# Autodesk Inventor assembly: Goldberg Assembly
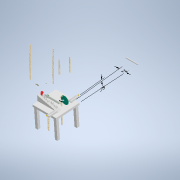
[picture p0: Inventor's stored thumbnail of the model, 180x180]
Saved by Autodesk Inventor 2021 (Build 250183000, 183)
## iProperties
Created: 2021-02-17
Part Number: Goldberg Assembly
Document SubType Name: Assembly
Designer: david
Author: david
## Documents named in this file (17)
- C:\Users\david\OneDrive\Documents\Inventor\Goldberg Assembly.iam
- C:\Users\david\OneDrive\Documents\Inventor\Tabl 12x12.ipt
- C:\Users\david\OneDrive\Documents\Inventor\Ball Ramp - Goldberg.ipt
- C:\Users\david\OneDrive\Documents\Inventor\Ball sphere - goldberg.ipt
- C:\Users\david\OneDrive\Documents\Inventor\Domino ramp.ipt
- C:\Users\david\OneDrive\Documents\Inventor\Domino.ipt
- C:\Users\david\OneDrive\Documents\Inventor\Cup- red.ipt
- C:\Users\david\OneDrive\Documents\Inventor\Inventor_2013_VEX_KOP_-_Imperial\Imperial\Motion\36 Tooth Gear.ipt
- C:\Users\david\OneDrive\Documents\Inventor\Inventor_2013_VEX_KOP_-_Imperial\Imperial\Motion\Shaft 2 inch.ipt
- C:\Users\david\OneDrive\Documents\Inventor\Inventor_2013_VEX_KOP_-_Imperial\Imperial\Motion\High Strength 6 Tooth Sprocket.ipt
- C:\Users\david\OneDrive\Documents\Inventor\Inventor_2013_VEX_KOP_-_Imperial\Imperial\Motion\High Strength 30 Tooth Sprocket.ipt
- C:\Users\david\OneDrive\Documents\Inventor\Inventor_2013_VEX_KOP_-_Imperial\Imperial\Motion\Chain Link.ipt
- C:\Users\david\OneDrive\Documents\Inventor\Inventor_2013_VEX_KOP_-_Imperial\Imperial\Motion\High Strength Chain Link.ipt
- C:\Users\david\OneDrive\Documents\Inventor\Inventor_2013_VEX_KOP_-_Imperial\Imperial\Motion\Tank Tread Traction Link.ipt
- C:\Users\david\OneDrive\Documents\Inventor\Inventor_2013_VEX_KOP_-_Imperial\Imperial\Structure\Chassis Bumper 15 Hole.ipt
- C:\Users\david\OneDrive\Documents\Inventor\Inventor_2013_VEX_KOP_-_Imperial\Imperial\Motion\Bearing Flat.ipt
- C:\Users\david\OneDrive\Documents\stick.ipt
## Components (228 placed, 16 different names)
1. Tabl 12x12:1 — Mate:1, Flush:1, Mate:2, Mate:3, Flush:2, Flush:3, Mate:22, Flush:4
2. Ball Ramp - Goldberg:1 — Mate:3, Mate:4, Flush:2, Tangent:1
3. Ball Ramp - Goldberg:2 — Mate:2, Tangent:2
4. Ball sphere - goldberg:1 — Tangent:1
5. Ball sphere - goldberg:2 — Tangent:2
6. Domino ramp:1 — Mate:1, Flush:1, Mate:4, Flush:3, Mate:5, Mate:6, Mate:7, Mate:8, Mate:9, Mate:10, Mate:11, Mate:12, Mate:13, Mate:14, Mate:15, Mate:16, Mate:17, Mate:18, Mate:20, Mate:21
7. Domino:1 — Mate:5
8. Domino:2 — Mate:7
9. Domino:3 — Mate:8
10. Domino:4 — Mate:6
11. Domino:5 — Mate:9
12. Domino:6 — Mate:10
13. Domino:7 — Mate:12
14. Domino:8 — Mate:15
15. Domino:9 — Mate:14
16. Domino:10 — Mate:11
17. Domino:11 — Mate:13
18. Cup- red:1 — Mate:16
19. Domino:12 — Mate:17
20. Domino:13 — Mate:18
21. 36 Tooth Gear:1 — Insert:81
22. Shaft 2 inch:1 — Mate:20, Insert:81, Insert:82
23. High Strength 6 Tooth Sprocket:1 — Mate:19, Insert:2, Insert:82
24. High Strength 30 Tooth Sprocket:1 — Mate:25, Mate:26, Mate:27, Mate:28, Mate:29
25. Chain Link:1
26. High Strength Chain Link:1 — Insert:1, Insert:2, Insert:276
27. High Strength Chain Link:3 — Insert:1, Mate:19
28. Tank Tread Traction Link:1
29. High Strength Chain Link:4 — Insert:9, Insert:10
30. High Strength Chain Link:10 — Insert:6, Insert:7, Insert:8, Insert:18
31. High Strength Chain Link:15 — Insert:11
32. High Strength Chain Link:21 — Insert:6, Insert:7, Insert:8, Insert:9
33. High Strength Chain Link:28 — Insert:10, Insert:11
34. High Strength Chain Link:31
35. High Strength Chain Link:32 — Insert:32
36. High Strength Chain Link:33 — Insert:18
37. High Strength Chain Link:34
38. High Strength Chain Link:35
39. High Strength Chain Link:36
40. High Strength Chain Link:37
41. High Strength Chain Link:38 — Insert:32
42. High Strength Chain Link:39
43. High Strength Chain Link:40
44. High Strength Chain Link:41
45. High Strength Chain Link:42 — Insert:110
46. High Strength Chain Link:43
47. High Strength Chain Link:44
48. High Strength Chain Link:45
49. High Strength Chain Link:46
50. High Strength Chain Link:47
51. High Strength Chain Link:48
52. High Strength Chain Link:49
53. High Strength Chain Link:50
54. High Strength Chain Link:51
55. High Strength Chain Link:52
56. High Strength Chain Link:53
57. High Strength Chain Link:54
58. High Strength Chain Link:55
59. High Strength Chain Link:56
60. High Strength Chain Link:57
61. High Strength Chain Link:58
62. High Strength Chain Link:59
63. High Strength Chain Link:60
64. High Strength Chain Link:61
65. High Strength Chain Link:62
66. High Strength Chain Link:63
67. High Strength Chain Link:64
68. High Strength Chain Link:65
69. High Strength Chain Link:66
70. High Strength Chain Link:67
71. High Strength Chain Link:68
72. High Strength Chain Link:69
73. High Strength Chain Link:70
74. High Strength Chain Link:71
75. High Strength Chain Link:72
76. High Strength Chain Link:73
77. High Strength Chain Link:74
78. High Strength Chain Link:75
79. High Strength Chain Link:76
80. High Strength Chain Link:77
81. High Strength Chain Link:78
82. High Strength Chain Link:79
83. High Strength Chain Link:80
84. High Strength Chain Link:81
85. High Strength Chain Link:82 — Insert:110
86. High Strength Chain Link:83
87. High Strength Chain Link:84
88. High Strength Chain Link:85
89. High Strength Chain Link:86
90. High Strength Chain Link:87
91. High Strength Chain Link:88
92. High Strength Chain Link:89
93. High Strength Chain Link:90
94. High Strength Chain Link:91
95. High Strength Chain Link:92
96. High Strength Chain Link:93
97. High Strength Chain Link:94
98. High Strength Chain Link:95
99. High Strength Chain Link:96
100. High Strength Chain Link:97
101. High Strength Chain Link:98
102. High Strength Chain Link:99
103. High Strength Chain Link:100
104. High Strength Chain Link:101
105. High Strength Chain Link:102
106. High Strength Chain Link:103
107. High Strength Chain Link:104
108. High Strength Chain Link:105
109. High Strength Chain Link:106
110. High Strength Chain Link:107
111. High Strength Chain Link:108
112. High Strength Chain Link:109
113. High Strength Chain Link:110
114. High Strength Chain Link:111
115. High Strength Chain Link:112
116. High Strength Chain Link:113
117. High Strength Chain Link:114
118. High Strength Chain Link:115
119. High Strength Chain Link:116
120. High Strength Chain Link:117
121. High Strength Chain Link:118
122. High Strength Chain Link:119
123. High Strength Chain Link:120
124. High Strength Chain Link:121
125. High Strength Chain Link:122
126. High Strength Chain Link:123
127. High Strength Chain Link:124
128. High Strength Chain Link:125
129. High Strength Chain Link:126
130. High Strength Chain Link:127
131. High Strength Chain Link:128
132. High Strength Chain Link:129
133. High Strength Chain Link:130
134. High Strength Chain Link:131
135. High Strength Chain Link:132
136. High Strength Chain Link:133
137. High Strength Chain Link:134
138. High Strength Chain Link:135
139. High Strength Chain Link:136 — Insert:276
140. High Strength Chain Link:137
141. High Strength Chain Link:138
142. High Strength Chain Link:139
143. High Strength Chain Link:140
144. High Strength Chain Link:141
145. High Strength Chain Link:142
146. High Strength Chain Link:143
147. High Strength Chain Link:144
148. High Strength Chain Link:145
149. High Strength Chain Link:146
150. High Strength Chain Link:147
151. High Strength Chain Link:148
152. High Strength Chain Link:149
153. High Strength Chain Link:150
154. High Strength Chain Link:151
155. High Strength Chain Link:152
156. High Strength Chain Link:153
157. High Strength Chain Link:154
158. High Strength Chain Link:155
159. High Strength Chain Link:156
160. High Strength Chain Link:157
161. High Strength Chain Link:158
162. High Strength Chain Link:159
163. High Strength Chain Link:160
164. High Strength Chain Link:161
165. High Strength Chain Link:162
166. High Strength Chain Link:163
167. High Strength Chain Link:164
168. High Strength Chain Link:165
169. High Strength Chain Link:166
170. High Strength Chain Link:167
171. High Strength Chain Link:168
172. High Strength Chain Link:169
173. High Strength Chain Link:170
174. High Strength Chain Link:171
175. High Strength Chain Link:172
176. High Strength Chain Link:173
177. High Strength Chain Link:174
178. High Strength Chain Link:175
179. High Strength Chain Link:176
180. High Strength Chain Link:177
181. High Strength Chain Link:178
182. High Strength Chain Link:179
183. High Strength Chain Link:180
184. High Strength Chain Link:181
185. High Strength Chain Link:182
186. High Strength Chain Link:183
187. High Strength Chain Link:184
188. High Strength Chain Link:185
189. High Strength Chain Link:186
190. High Strength Chain Link:187
191. High Strength Chain Link:188
192. High Strength Chain Link:189
193. High Strength Chain Link:190
194. High Strength Chain Link:191
195. High Strength Chain Link:192
196. High Strength Chain Link:193
197. High Strength Chain Link:194
198. High Strength Chain Link:195
199. High Strength Chain Link:196
200. High Strength Chain Link:197
201. High Strength Chain Link:198
202. High Strength Chain Link:199
203. High Strength Chain Link:200
204. High Strength Chain Link:201
205. High Strength Chain Link:202
206. High Strength Chain Link:203
207. High Strength Chain Link:204
208. High Strength Chain Link:205
209. High Strength Chain Link:206
210. High Strength Chain Link:207
211. High Strength Chain Link:208
212. High Strength Chain Link:209
213. High Strength Chain Link:210
214. High Strength Chain Link:211 — Mate:28
215. High Strength Chain Link:212
216. High Strength Chain Link:213 — Mate:29, Mate:30
217. High Strength Chain Link:214
218. High Strength Chain Link:215 — Mate:27
219. High Strength Chain Link:216
220. High Strength Chain Link:217 — Mate:30
221. High Strength Chain Link:218
222. High Strength Chain Link:219 — Mate:26
223. Chassis Bumper 15 Hole:1 — Mate:21, Mate:22, Flush:4, Mate:23, Mate:24, Flush:5
224. Shaft 2 inch:2 — Mate:23, Mate:24, Flush:5, Insert:277
225. Bearing Flat:1 — Insert:277, Mate:25
226. stick:1
227. stick:2
228. stick:3
## Relationships (311: Insert 274, Mate 30, Flush 5, Tangent 2)
- Mate:1: Tabl 12x12:1 ↔ Domino ramp:1
- Flush:1 (203.2 mm): Tabl 12x12:1 ↔ Domino ramp:1
- Mate:2: Tabl 12x12:1 ↔ Ball Ramp - Goldberg:2
- Mate:3: Tabl 12x12:1 ↔ Ball Ramp - Goldberg:1
- Mate:4: Ball Ramp - Goldberg:1 ↔ Domino ramp:1
- Flush:2 (50.8 mm): Tabl 12x12:1 ↔ Ball Ramp - Goldberg:1
- Flush:3: Tabl 12x12:1 ↔ Domino ramp:1
- Mate:5: Domino ramp:1 ↔ Domino:1
- Mate:6: Domino ramp:1 ↔ Domino:4
- Mate:7: Domino ramp:1 ↔ Domino:2
- Mate:8: Domino ramp:1 ↔ Domino:3
- Mate:9: Domino ramp:1 ↔ Domino:5
- Mate:10: Domino ramp:1 ↔ Domino:6
- Mate:11: Domino ramp:1 ↔ Domino:10
- Mate:12: Domino ramp:1 ↔ Domino:7
- Mate:13: Domino ramp:1 ↔ Domino:11
- Mate:14: Domino ramp:1 ↔ Domino:9
- Mate:15: Domino ramp:1 ↔ Domino:8
- Mate:16: Domino ramp:1 ↔ Cup- red:1
- Mate:17: Domino ramp:1 ↔ Domino:12
- Mate:18: Domino ramp:1 ↔ Domino:13
- Tangent:1: Ball Ramp - Goldberg:1 ↔ Ball sphere - goldberg:1
- Tangent:2: Ball Ramp - Goldberg:2 ↔ Ball sphere - goldberg:2
- Insert:1: High Strength Chain Link:1 ↔ High Strength Chain Link:3
- Mate:19: High Strength 6 Tooth Sprocket:1 ↔ High Strength Chain Link:3
- Insert:2: High Strength 6 Tooth Sprocket:1 ↔ High Strength Chain Link:1
- Insert:6: High Strength Chain Link:10 ↔ High Strength Chain Link:21
- Insert:7: High Strength Chain Link:10 ↔ High Strength Chain Link:21
- Insert:8: High Strength Chain Link:10 ↔ High Strength Chain Link:21
- Insert:9: High Strength Chain Link:4 ↔ High Strength Chain Link:21
- Insert:10: High Strength Chain Link:4 ↔ High Strength Chain Link:28
- Insert:11: High Strength Chain Link:15 ↔ High Strength Chain Link:28
- [Insert]: High Strength Chain Link:32 ↔ High Strength Chain Link:34
- [Insert]: High Strength Chain Link:32 ↔ High Strength Chain Link:34
- [Insert]: High Strength Chain Link:32 ↔ High Strength Chain Link:34
- [Insert]: High Strength Chain Link:31 ↔ High Strength Chain Link:34
- [Insert]: High Strength Chain Link:31 ↔ High Strength Chain Link:35
- [Insert]: High Strength Chain Link:33 ↔ High Strength Chain Link:35
- Insert:18: High Strength Chain Link:10 ↔ High Strength Chain Link:33
- [Insert]: High Strength Chain Link:37 ↔ High Strength Chain Link:39
- [Insert]: High Strength Chain Link:37 ↔ High Strength Chain Link:39
- [Insert]: High Strength Chain Link:37 ↔ High Strength Chain Link:39
- [Insert]: High Strength Chain Link:36 ↔ High Strength Chain Link:39
- [Insert]: High Strength Chain Link:36 ↔ High Strength Chain Link:40
- [Insert]: High Strength Chain Link:38 ↔ High Strength Chain Link:40
- [Insert]: High Strength Chain Link:42 ↔ High Strength Chain Link:44
- [Insert]: High Strength Chain Link:42 ↔ High Strength Chain Link:44
- [Insert]: High Strength Chain Link:42 ↔ High Strength Chain Link:44
- [Insert]: High Strength Chain Link:41 ↔ High Strength Chain Link:44
- [Insert]: High Strength Chain Link:41 ↔ High Strength Chain Link:45
- [Insert]: High Strength Chain Link:43 ↔ High Strength Chain Link:45
- [Insert]: High Strength Chain Link:37 ↔ High Strength Chain Link:43
- Insert:32: High Strength Chain Link:32 ↔ High Strength Chain Link:38
- [Insert]: High Strength Chain Link:46 ↔ High Strength Chain Link:47
- [Insert]: High Strength Chain Link:46 ↔ High Strength Chain Link:47
- [Insert]: High Strength Chain Link:46 ↔ High Strength Chain Link:47
- [Insert]: High Strength Chain Link:49 ↔ High Strength Chain Link:51
- [Insert]: High Strength Chain Link:49 ↔ High Strength Chain Link:51
- [Insert]: High Strength Chain Link:49 ↔ High Strength Chain Link:51
- [Insert]: High Strength Chain Link:48 ↔ High Strength Chain Link:51
- [Insert]: High Strength Chain Link:48 ↔ High Strength Chain Link:52
- [Insert]: High Strength Chain Link:50 ↔ High Strength Chain Link:52
- [Insert]: High Strength Chain Link:46 ↔ High Strength Chain Link:50
- [Insert]: High Strength Chain Link:54 ↔ High Strength Chain Link:56
- [Insert]: High Strength Chain Link:54 ↔ High Strength Chain Link:56
- [Insert]: High Strength Chain Link:54 ↔ High Strength Chain Link:56
- [Insert]: High Strength Chain Link:53 ↔ High Strength Chain Link:56
- [Insert]: High Strength Chain Link:53 ↔ High Strength Chain Link:57
- [Insert]: High Strength Chain Link:55 ↔ High Strength Chain Link:57
- [Insert]: High Strength Chain Link:59 ↔ High Strength Chain Link:61
- [Insert]: High Strength Chain Link:59 ↔ High Strength Chain Link:61
- [Insert]: High Strength Chain Link:59 ↔ High Strength Chain Link:61
- [Insert]: High Strength Chain Link:58 ↔ High Strength Chain Link:61
- [Insert]: High Strength Chain Link:58 ↔ High Strength Chain Link:62
- [Insert]: High Strength Chain Link:60 ↔ High Strength Chain Link:62
- [Insert]: High Strength Chain Link:54 ↔ High Strength Chain Link:60
- [Insert]: High Strength Chain Link:49 ↔ High Strength Chain Link:55
- [Insert]: High Strength Chain Link:63 ↔ High Strength Chain Link:64
- [Insert]: High Strength Chain Link:63 ↔ High Strength Chain Link:64
- [Insert]: High Strength Chain Link:63 ↔ High Strength Chain Link:64
- [Insert]: High Strength Chain Link:66 ↔ High Strength Chain Link:68
- [Insert]: High Strength Chain Link:66 ↔ High Strength Chain Link:68
- [Insert]: High Strength Chain Link:66 ↔ High Strength Chain Link:68
- [Insert]: High Strength Chain Link:65 ↔ High Strength Chain Link:68
- [Insert]: High Strength Chain Link:65 ↔ High Strength Chain Link:69
- [Insert]: High Strength Chain Link:67 ↔ High Strength Chain Link:69
- [Insert]: High Strength Chain Link:63 ↔ High Strength Chain Link:67
- [Insert]: High Strength Chain Link:71 ↔ High Strength Chain Link:73
- [Insert]: High Strength Chain Link:71 ↔ High Strength Chain Link:73
- [Insert]: High Strength Chain Link:71 ↔ High Strength Chain Link:73
- [Insert]: High Strength Chain Link:70 ↔ High Strength Chain Link:73
- [Insert]: High Strength Chain Link:70 ↔ High Strength Chain Link:74
- [Insert]: High Strength Chain Link:72 ↔ High Strength Chain Link:74
- [Insert]: High Strength Chain Link:76 ↔ High Strength Chain Link:78
- [Insert]: High Strength Chain Link:76 ↔ High Strength Chain Link:78
- [Insert]: High Strength Chain Link:76 ↔ High Strength Chain Link:78
- [Insert]: High Strength Chain Link:75 ↔ High Strength Chain Link:78
- [Insert]: High Strength Chain Link:75 ↔ High Strength Chain Link:79
- [Insert]: High Strength Chain Link:77 ↔ High Strength Chain Link:79
- [Insert]: High Strength Chain Link:71 ↔ High Strength Chain Link:77
- [Insert]: High Strength Chain Link:66 ↔ High Strength Chain Link:72
- Mate:20: Domino ramp:1 ↔ Shaft 2 inch:1
- Insert:81 (-31.75 mm): 36 Tooth Gear:1 ↔ Shaft 2 inch:1
- Insert:82 (-6.35 mm): Shaft 2 inch:1 ↔ High Strength 6 Tooth Sprocket:1
- [Insert]: High Strength Chain Link:81 ↔ High Strength Chain Link:83
- [Insert]: High Strength Chain Link:81 ↔ High Strength Chain Link:83
- [Insert]: High Strength Chain Link:81 ↔ High Strength Chain Link:83
- [Insert]: High Strength Chain Link:80 ↔ High Strength Chain Link:83
- [Insert]: High Strength Chain Link:80 ↔ High Strength Chain Link:84
- [Insert]: High Strength Chain Link:82 ↔ High Strength Chain Link:84
- [Insert]: High Strength Chain Link:86 ↔ High Strength Chain Link:88
- [Insert]: High Strength Chain Link:86 ↔ High Strength Chain Link:88
- [Insert]: High Strength Chain Link:86 ↔ High Strength Chain Link:88
- [Insert]: High Strength Chain Link:85 ↔ High Strength Chain Link:88
- [Insert]: High Strength Chain Link:85 ↔ High Strength Chain Link:89
- [Insert]: High Strength Chain Link:87 ↔ High Strength Chain Link:89
- [Insert]: High Strength Chain Link:81 ↔ High Strength Chain Link:87
- [Insert]: High Strength Chain Link:91 ↔ High Strength Chain Link:93
- [Insert]: High Strength Chain Link:91 ↔ High Strength Chain Link:93
- [Insert]: High Strength Chain Link:91 ↔ High Strength Chain Link:93
- [Insert]: High Strength Chain Link:90 ↔ High Strength Chain Link:93
- [Insert]: High Strength Chain Link:90 ↔ High Strength Chain Link:94
- [Insert]: High Strength Chain Link:92 ↔ High Strength Chain Link:94
- [Insert]: High Strength Chain Link:96 ↔ High Strength Chain Link:98
- [Insert]: High Strength Chain Link:96 ↔ High Strength Chain Link:98
- [Insert]: High Strength Chain Link:96 ↔ High Strength Chain Link:98
- [Insert]: High Strength Chain Link:95 ↔ High Strength Chain Link:98
- [Insert]: High Strength Chain Link:95 ↔ High Strength Chain Link:99
- [Insert]: High Strength Chain Link:97 ↔ High Strength Chain Link:99
- [Insert]: High Strength Chain Link:91 ↔ High Strength Chain Link:97
- [Insert]: High Strength Chain Link:86 ↔ High Strength Chain Link:92
- Insert:110: High Strength Chain Link:42 ↔ High Strength Chain Link:82
- [Insert]: High Strength Chain Link:101 ↔ High Strength Chain Link:103
- [Insert]: High Strength Chain Link:101 ↔ High Strength Chain Link:103
- [Insert]: High Strength Chain Link:101 ↔ High Strength Chain Link:103
- [Insert]: High Strength Chain Link:100 ↔ High Strength Chain Link:103
- [Insert]: High Strength Chain Link:100 ↔ High Strength Chain Link:104
- [Insert]: High Strength Chain Link:102 ↔ High Strength Chain Link:104
- [Insert]: High Strength Chain Link:106 ↔ High Strength Chain Link:108
- [Insert]: High Strength Chain Link:106 ↔ High Strength Chain Link:108
- [Insert]: High Strength Chain Link:106 ↔ High Strength Chain Link:108
- [Insert]: High Strength Chain Link:105 ↔ High Strength Chain Link:108
- [Insert]: High Strength Chain Link:105 ↔ High Strength Chain Link:109
- [Insert]: High Strength Chain Link:107 ↔ High Strength Chain Link:109
- [Insert]: High Strength Chain Link:101 ↔ High Strength Chain Link:107
- [Insert]: High Strength Chain Link:111 ↔ High Strength Chain Link:113
- [Insert]: High Strength Chain Link:111 ↔ High Strength Chain Link:113
- [Insert]: High Strength Chain Link:111 ↔ High Strength Chain Link:113
- [Insert]: High Strength Chain Link:110 ↔ High Strength Chain Link:113
- [Insert]: High Strength Chain Link:110 ↔ High Strength Chain Link:114
- [Insert]: High Strength Chain Link:112 ↔ High Strength Chain Link:114
- [Insert]: High Strength Chain Link:116 ↔ High Strength Chain Link:118
- [Insert]: High Strength Chain Link:116 ↔ High Strength Chain Link:118
- [Insert]: High Strength Chain Link:116 ↔ High Strength Chain Link:118
- [Insert]: High Strength Chain Link:115 ↔ High Strength Chain Link:118
- [Insert]: High Strength Chain Link:115 ↔ High Strength Chain Link:119
- [Insert]: High Strength Chain Link:117 ↔ High Strength Chain Link:119
- [Insert]: High Strength Chain Link:111 ↔ High Strength Chain Link:117
- [Insert]: High Strength Chain Link:106 ↔ High Strength Chain Link:112
- [Insert]: High Strength Chain Link:121 ↔ High Strength Chain Link:123
- [Insert]: High Strength Chain Link:121 ↔ High Strength Chain Link:123
- [Insert]: High Strength Chain Link:121 ↔ High Strength Chain Link:123
- [Insert]: High Strength Chain Link:120 ↔ High Strength Chain Link:123
- [Insert]: High Strength Chain Link:120 ↔ High Strength Chain Link:124
- [Insert]: High Strength Chain Link:122 ↔ High Strength Chain Link:124
- [Insert]: High Strength Chain Link:126 ↔ High Strength Chain Link:128
- [Insert]: High Strength Chain Link:126 ↔ High Strength Chain Link:128
- [Insert]: High Strength Chain Link:126 ↔ High Strength Chain Link:128
- [Insert]: High Strength Chain Link:125 ↔ High Strength Chain Link:128
- [Insert]: High Strength Chain Link:125 ↔ High Strength Chain Link:129
- [Insert]: High Strength Chain Link:127 ↔ High Strength Chain Link:129
- [Insert]: High Strength Chain Link:121 ↔ High Strength Chain Link:127
- [Insert]: High Strength Chain Link:131 ↔ High Strength Chain Link:133
- [Insert]: High Strength Chain Link:131 ↔ High Strength Chain Link:133
- [Insert]: High Strength Chain Link:131 ↔ High Strength Chain Link:133
- [Insert]: High Strength Chain Link:130 ↔ High Strength Chain Link:133
- [Insert]: High Strength Chain Link:130 ↔ High Strength Chain Link:134
- [Insert]: High Strength Chain Link:132 ↔ High Strength Chain Link:134
- [Insert]: High Strength Chain Link:136 ↔ High Strength Chain Link:138
- [Insert]: High Strength Chain Link:136 ↔ High Strength Chain Link:138
- [Insert]: High Strength Chain Link:136 ↔ High Strength Chain Link:138
- [Insert]: High Strength Chain Link:135 ↔ High Strength Chain Link:138
- [Insert]: High Strength Chain Link:135 ↔ High Strength Chain Link:139
- [Insert]: High Strength Chain Link:137 ↔ High Strength Chain Link:139
- [Insert]: High Strength Chain Link:131 ↔ High Strength Chain Link:137
- [Insert]: High Strength Chain Link:126 ↔ High Strength Chain Link:132
- [Insert]: High Strength Chain Link:116 ↔ High Strength Chain Link:122
- [Insert]: High Strength Chain Link:141 ↔ High Strength Chain Link:143
- [Insert]: High Strength Chain Link:141 ↔ High Strength Chain Link:143
- [Insert]: High Strength Chain Link:141 ↔ High Strength Chain Link:143
- [Insert]: High Strength Chain Link:140 ↔ High Strength Chain Link:143
- [Insert]: High Strength Chain Link:140 ↔ High Strength Chain Link:144
- [Insert]: High Strength Chain Link:142 ↔ High Strength Chain Link:144
- [Insert]: High Strength Chain Link:146 ↔ High Strength Chain Link:148
- [Insert]: High Strength Chain Link:146 ↔ High Strength Chain Link:148
- [Insert]: High Strength Chain Link:146 ↔ High Strength Chain Link:148
- [Insert]: High Strength Chain Link:145 ↔ High Strength Chain Link:148
- [Insert]: High Strength Chain Link:145 ↔ High Strength Chain Link:149
- [Insert]: High Strength Chain Link:147 ↔ High Strength Chain Link:149
- [Insert]: High Strength Chain Link:141 ↔ High Strength Chain Link:147
- [Insert]: High Strength Chain Link:151 ↔ High Strength Chain Link:153
- [Insert]: High Strength Chain Link:151 ↔ High Strength Chain Link:153
- [Insert]: High Strength Chain Link:151 ↔ High Strength Chain Link:153
- [Insert]: High Strength Chain Link:150 ↔ High Strength Chain Link:153
- [Insert]: High Strength Chain Link:150 ↔ High Strength Chain Link:154
- [Insert]: High Strength Chain Link:152 ↔ High Strength Chain Link:154
- [Insert]: High Strength Chain Link:156 ↔ High Strength Chain Link:158
- [Insert]: High Strength Chain Link:156 ↔ High Strength Chain Link:158
- [Insert]: High Strength Chain Link:156 ↔ High Strength Chain Link:158
- [Insert]: High Strength Chain Link:155 ↔ High Strength Chain Link:158
- [Insert]: High Strength Chain Link:155 ↔ High Strength Chain Link:159
- [Insert]: High Strength Chain Link:157 ↔ High Strength Chain Link:159
- [Insert]: High Strength Chain Link:151 ↔ High Strength Chain Link:157
- [Insert]: High Strength Chain Link:146 ↔ High Strength Chain Link:152
- [Insert]: High Strength Chain Link:161 ↔ High Strength Chain Link:163
- [Insert]: High Strength Chain Link:161 ↔ High Strength Chain Link:163
- [Insert]: High Strength Chain Link:161 ↔ High Strength Chain Link:163
- [Insert]: High Strength Chain Link:160 ↔ High Strength Chain Link:163
- [Insert]: High Strength Chain Link:160 ↔ High Strength Chain Link:164
- [Insert]: High Strength Chain Link:162 ↔ High Strength Chain Link:164
- [Insert]: High Strength Chain Link:166 ↔ High Strength Chain Link:168
- [Insert]: High Strength Chain Link:166 ↔ High Strength Chain Link:168
- [Insert]: High Strength Chain Link:166 ↔ High Strength Chain Link:168
- [Insert]: High Strength Chain Link:165 ↔ High Strength Chain Link:168
- [Insert]: High Strength Chain Link:165 ↔ High Strength Chain Link:169
- [Insert]: High Strength Chain Link:167 ↔ High Strength Chain Link:169
- [Insert]: High Strength Chain Link:161 ↔ High Strength Chain Link:167
- [Insert]: High Strength Chain Link:171 ↔ High Strength Chain Link:173
- [Insert]: High Strength Chain Link:171 ↔ High Strength Chain Link:173
- [Insert]: High Strength Chain Link:171 ↔ High Strength Chain Link:173
- [Insert]: High Strength Chain Link:170 ↔ High Strength Chain Link:173
- [Insert]: High Strength Chain Link:170 ↔ High Strength Chain Link:174
- [Insert]: High Strength Chain Link:172 ↔ High Strength Chain Link:174
- [Insert]: High Strength Chain Link:176 ↔ High Strength Chain Link:178
- [Insert]: High Strength Chain Link:176 ↔ High Strength Chain Link:178
- [Insert]: High Strength Chain Link:176 ↔ High Strength Chain Link:178
- [Insert]: High Strength Chain Link:175 ↔ High Strength Chain Link:178
- [Insert]: High Strength Chain Link:175 ↔ High Strength Chain Link:179
- [Insert]: High Strength Chain Link:177 ↔ High Strength Chain Link:179
- [Insert]: High Strength Chain Link:171 ↔ High Strength Chain Link:177
- [Insert]: High Strength Chain Link:166 ↔ High Strength Chain Link:172
- [Insert]: High Strength Chain Link:156 ↔ High Strength Chain Link:162
- [Insert]: High Strength Chain Link:181 ↔ High Strength Chain Link:183
- [Insert]: High Strength Chain Link:181 ↔ High Strength Chain Link:183
- [Insert]: High Strength Chain Link:181 ↔ High Strength Chain Link:183
- [Insert]: High Strength Chain Link:180 ↔ High Strength Chain Link:183
- [Insert]: High Strength Chain Link:180 ↔ High Strength Chain Link:184
- [Insert]: High Strength Chain Link:182 ↔ High Strength Chain Link:184
- [Insert]: High Strength Chain Link:186 ↔ High Strength Chain Link:188
- [Insert]: High Strength Chain Link:186 ↔ High Strength Chain Link:188
- [Insert]: High Strength Chain Link:186 ↔ High Strength Chain Link:188
- [Insert]: High Strength Chain Link:185 ↔ High Strength Chain Link:188
- [Insert]: High Strength Chain Link:185 ↔ High Strength Chain Link:189
- [Insert]: High Strength Chain Link:187 ↔ High Strength Chain Link:189
- [Insert]: High Strength Chain Link:181 ↔ High Strength Chain Link:187
- [Insert]: High Strength Chain Link:191 ↔ High Strength Chain Link:193
- [Insert]: High Strength Chain Link:191 ↔ High Strength Chain Link:193
- [Insert]: High Strength Chain Link:191 ↔ High Strength Chain Link:193
- [Insert]: High Strength Chain Link:190 ↔ High Strength Chain Link:193
- [Insert]: High Strength Chain Link:190 ↔ High Strength Chain Link:194
- [Insert]: High Strength Chain Link:192 ↔ High Strength Chain Link:194
- [Insert]: High Strength Chain Link:196 ↔ High Strength Chain Link:198
- [Insert]: High Strength Chain Link:196 ↔ High Strength Chain Link:198
- [Insert]: High Strength Chain Link:196 ↔ High Strength Chain Link:198
- [Insert]: High Strength Chain Link:195 ↔ High Strength Chain Link:198
- [Insert]: High Strength Chain Link:195 ↔ High Strength Chain Link:199
- [Insert]: High Strength Chain Link:197 ↔ High Strength Chain Link:199
- [Insert]: High Strength Chain Link:191 ↔ High Strength Chain Link:197
- [Insert]: High Strength Chain Link:186 ↔ High Strength Chain Link:192
- [Insert]: High Strength Chain Link:201 ↔ High Strength Chain Link:203
- [Insert]: High Strength Chain Link:201 ↔ High Strength Chain Link:203
- [Insert]: High Strength Chain Link:201 ↔ High Strength Chain Link:203
- [Insert]: High Strength Chain Link:200 ↔ High Strength Chain Link:203
- [Insert]: High Strength Chain Link:200 ↔ High Strength Chain Link:204
- [Insert]: High Strength Chain Link:202 ↔ High Strength Chain Link:204
- [Insert]: High Strength Chain Link:206 ↔ High Strength Chain Link:208
- [Insert]: High Strength Chain Link:206 ↔ High Strength Chain Link:208
- [Insert]: High Strength Chain Link:206 ↔ High Strength Chain Link:208
- [Insert]: High Strength Chain Link:205 ↔ High Strength Chain Link:208
- [Insert]: High Strength Chain Link:205 ↔ High Strength Chain Link:209
- [Insert]: High Strength Chain Link:207 ↔ High Strength Chain Link:209
- [Insert]: High Strength Chain Link:201 ↔ High Strength Chain Link:207
- [Insert]: High Strength Chain Link:211 ↔ High Strength Chain Link:213
- [Insert]: High Strength Chain Link:211 ↔ High Strength Chain Link:213
- [Insert]: High Strength Chain Link:211 ↔ High Strength Chain Link:213
- [Insert]: High Strength Chain Link:210 ↔ High Strength Chain Link:213
- [Insert]: High Strength Chain Link:210 ↔ High Strength Chain Link:214
- [Insert]: High Strength Chain Link:212 ↔ High Strength Chain Link:214
- [Insert]: High Strength Chain Link:216 ↔ High Strength Chain Link:218
- [Insert]: High Strength Chain Link:216 ↔ High Strength Chain Link:218
- [Insert]: High Strength Chain Link:216 ↔ High Strength Chain Link:218
- [Insert]: High Strength Chain Link:215 ↔ High Strength Chain Link:218
- [Insert]: High Strength Chain Link:215 ↔ High Strength Chain Link:219
- [Insert]: High Strength Chain Link:217 ↔ High Strength Chain Link:219
- [Insert]: High Strength Chain Link:211 ↔ High Strength Chain Link:217
- [Insert]: High Strength Chain Link:206 ↔ High Strength Chain Link:212
- [Insert]: High Strength Chain Link:196 ↔ High Strength Chain Link:202
- Insert:276: High Strength Chain Link:1 ↔ High Strength Chain Link:136
- Mate:21: Domino ramp:1 ↔ Chassis Bumper 15 Hole:1
- Mate:22 (50.8 mm): Tabl 12x12:1 ↔ Chassis Bumper 15 Hole:1
- Flush:4 (76.2 mm): Tabl 12x12:1 ↔ Chassis Bumper 15 Hole:1
- Mate:23: Chassis Bumper 15 Hole:1 ↔ Shaft 2 inch:2
- Mate:24: Chassis Bumper 15 Hole:1 ↔ Shaft 2 inch:2
- Flush:5 (-12.7 mm): Chassis Bumper 15 Hole:1 ↔ Shaft 2 inch:2
- Insert:277 (-12.7 mm): Shaft 2 inch:2 ↔ Bearing Flat:1
- Mate:25: High Strength 30 Tooth Sprocket:1 ↔ Bearing Flat:1
- Mate:26: High Strength 30 Tooth Sprocket:1 ↔ High Strength Chain Link:219
- Mate:27: High Strength 30 Tooth Sprocket:1 ↔ High Strength Chain Link:215
- Mate:28: High Strength 30 Tooth Sprocket:1 ↔ High Strength Chain Link:211
- Mate:29: High Strength 30 Tooth Sprocket:1 ↔ High Strength Chain Link:213
- Mate:30: High Strength Chain Link:213 ↔ High Strength Chain Link:217
## Named parameters: d46_d44 = 0 mm, d47_d45 = 0 mm, d48_d40 = 0 mm, d49_d41 = 0 mm, d50_d42 = 0 mm, d51_d43 = 0 mm, d53_d44 = 0 mm, d54_d45 = 0 mm, d55_d46_d44 = 0 mm, d56_d47_d45 = 0 mm, d57_d48_d40 = 0 mm, d58_d49_d41 = 0 mm, d59_d50_d42 = 0 mm, d60_d51_d43 = 0 mm, d61_d52 = 0 mm, d62_d40 = 0 mm, d63_d41 = 0 mm, d64_d42 = 0 mm, d65_d43 = 0 mm, d67_d46_d44 = 0 mm, d68_d47_d45 = 0 mm, d69_d48_d40 = 0 mm, d70_d49_d41 = 0 mm, d71_d50_d42 = 0 mm, d72_d51_d43 = 0 mm, d73_d52 = 0 mm, d74_d53_d44 = 0 mm, d75_d54_d45 = 0 mm, d76_d55_d46_d44 = 0 mm, d77_d56_d47_d45 = 0 mm, d78_d57_d48_d40 = 0 mm, d79_d58_d49_d41 = 0 mm, d80_d59_d50_d42 = 0 mm, d81_d60_d51_d43 = 0 mm, d82_d61_d52 = 0 mm, d83_d62_d40 = 0 mm, d84_d63_d41 = 0 mm, d85_d64_d42 = 0 mm, d86_d65_d43 = 0 mm, d87_d40 = 0 mm, d88_d41 = 0 mm, d89_d42 = 0 mm, d90_d66 = 0 mm, d91_d67_d46_d44 = 0 mm, d92_d68_d47_d45 = 0 mm, d93_d69_d48_d40 = 0 mm, d94_d70_d49_d41 = 0 mm, d95_d71_d50_d42 = 0 mm, d96_d72_d51_d43 = 0 mm, d97_d73_d52 = 0 mm, d98_d74_d53_d44 = 0 mm, d99_d75_d54_d45 = 0 mm, d100_d76_d55_d46_d44 = 0 mm, d101_d77_d56_d47_d45 = 0 mm, d102_d78_d57_d48_d40 = 0 mm, d103_d79_d58_d49_d41 = 0 mm, d104_d80_d59_d50_d42 = 0 mm, d105_d81_d60_d51_d43 = 0 mm, d106_d82_d61_d52 = 0 mm, d107_d83_d62_d40 = 0 mm, d108_d84_d63_d41 = 0 mm, d109_d85_d64_d42 = 0 mm, d110_d86_d65_d43 = 0 mm, d111_d87_d40 = 0 mm, d112_d88_d41 = 0 mm, d113_d89_d42 = 0 mm, d114_d90_d66 = 0 mm, d118_d44 = 0 mm, d119_d45 = 0 mm, d120_d46_d44 = 0 mm, d121_d47_d45 = 0 mm, d122_d48_d40 = 0 mm, d123_d49_d41 = 0 mm, d124_d50_d42 = 0 mm, d125_d51_d43 = 0 mm, d126_d52 = 0 mm, d127_d53_d44 = 0 mm, d128_d54_d45 = 0 mm, d129_d55_d46_d44 = 0 mm, d130_d56_d47_d45 = 0 mm, d131_d57_d48_d40 = 0 mm, d132_d58_d49_d41 = 0 mm, d133_d59_d50_d42 = 0 mm, d134_d60_d51_d43 = 0 mm, d135_d61_d52 = 0 mm, d136_d62_d40 = 0 mm, d137_d63_d41 = 0 mm, d138_d64_d42 = 0 mm, d139_d65_d43 = 0 mm, d140_d40 = 0 mm, d141_d41 = 0 mm, d142_d42 = 0 mm, d143_d43 = 0 mm, d144_d66 = 0 mm, d146_d145 = 0 mm, d147_d44 = 0 mm, d148_d45 = 0 mm, d149_d46_d44 = 0 mm, d150_d47_d45 = 0 mm, d151_d48_d40 = 0 mm, d152_d49_d41 = 0 mm, d153_d50_d42 = 0 mm, d154_d51_d43 = 0 mm, d155_d52 = 0 mm, d156_d53_d44 = 0 mm, d157_d54_d45 = 0 mm, d158_d55_d46_d44 = 0 mm, d159_d56_d47_d45 = 0 mm, d160_d57_d48_d40 = 0 mm, d161_d58_d49_d41 = 0 mm, d162_d59_d50_d42 = 0 mm, d163_d60_d51_d43 = 0 mm, d164_d61_d52 = 0 mm, d165_d62_d40 = 0 mm, d166_d63_d41 = 0 mm, d167_d64_d42 = 0 mm, d168_d65_d43 = 0 mm, d169_d40 = 0 mm, d170_d41 = 0 mm, d171_d42 = 0 mm, d172_d43 = 0 mm, d173_d118_d44 = 0 mm, d174_d119_d45 = 0 mm, d175_d120_d46_d44 = 0 mm, d176_d121_d47_d45 = 0 mm, d177_d122_d48_d40 = 0 mm, d178_d123_d49_d41 = 0 mm, d179_d124_d50_d42 = 0 mm, d180_d125_d51_d43 = 0 mm, d181_d126_d52 = 0 mm, d182_d127_d53_d44 = 0 mm, d183_d128_d54_d45 = 0 mm, d184_d129_d55_d46_d44 = 0 mm, d185_d130_d56_d47_d45 = 0 mm, d186_d131_d57_d48_d40 = 0 mm, d187_d132_d58_d49_d41 = 0 mm, d188_d133_d59_d50_d42 = 0 mm, d189_d134_d60_d51_d43 = 0 mm, d190_d135_d61_d52 = 0 mm, d191_d136_d62_d40 = 0 mm, d192_d137_d63_d41 = 0 mm, d193_d138_d64_d42 = 0 mm, d194_d139_d65_d43 = 0 mm, d195_d140_d40 = 0 mm, d196_d141_d41 = 0 mm, d197_d142_d42 = 0 mm, d198_d143_d43 = 0 mm, d199_d144_d66 = 0 mm, d200_d66 = 0 mm, d201_d145 = 0 mm, d202_d44 = 0 mm, d203_d45 = 0 mm, d204_d46_d44 = 0 mm, d205_d47_d45 = 0 mm, d206_d48_d40 = 0 mm, d207_d49_d41 = 0 mm, d208_d50_d42 = 0 mm, d209_d51_d43 = 0 mm, d210_d52 = 0 mm, d211_d53_d44 = 0 mm, d212_d54_d45 = 0 mm, d213_d55_d46_d44 = 0 mm, d214_d56_d47_d45 = 0 mm, d215_d57_d48_d40 = 0 mm, d216_d58_d49_d41 = 0 mm, d217_d59_d50_d42 = 0 mm, d218_d60_d51_d43 = 0 mm, d219_d61_d52 = 0 mm, d220_d62_d40 = 0 mm, d221_d63_d41 = 0 mm, d222_d64_d42 = 0 mm, d223_d65_d43 = 0 mm, d224_d40 = 0 mm, d225_d41 = 0 mm, d226_d42 = 0 mm, d227_d43 = 0 mm, d228_d118_d44 = 0 mm, d229_d119_d45 = 0 mm, d230_d120_d46_d44 = 0 mm, d231_d121_d47_d45 = 0 mm, d232_d122_d48_d40 = 0 mm, d233_d123_d49_d41 = 0 mm, d234_d124_d50_d42 = 0 mm, d235_d125_d51_d43 = 0 mm, d236_d126_d52 = 0 mm, d237_d127_d53_d44 = 0 mm, d238_d128_d54_d45 = 0 mm, d239_d129_d55_d46_d44 = 0 mm, d240_d130_d56_d47_d45 = 0 mm, d241_d131_d57_d48_d40 = 0 mm, d242_d132_d58_d49_d41 = 0 mm, d243_d133_d59_d50_d42 = 0 mm, d244_d134_d60_d51_d43 = 0 mm, d245_d135_d61_d52 = 0 mm, d246_d136_d62_d40 = 0 mm, d247_d137_d63_d41 = 0 mm, d248_d138_d64_d42 = 0 mm, d249_d139_d65_d43 = 0 mm, d250_d140_d40 = 0 mm, d251_d141_d41 = 0 mm, d252_d142_d42 = 0 mm, d253_d143_d43 = 0 mm, d254_d144_d66 = 0 mm, d255_d66 = 0 mm, d256_d145 = 0 mm, d257_d44 = 0 mm, d258_d45 = 0 mm, d259_d46_d44 = 0 mm, d260_d47_d45 = 0 mm, d261_d48_d40 = 0 mm, d262_d49_d41 = 0 mm, d263_d50_d42 = 0 mm, d264_d51_d43 = 0 mm, d265_d52 = 0 mm, d266_d53_d44 = 0 mm, d267_d54_d45 = 0 mm, d268_d55_d46_d44 = 0 mm, d269_d56_d47_d45 = 0 mm, d270_d57_d48_d40 = 0 mm, d271_d58_d49_d41 = 0 mm, d272_d59_d50_d42 = 0 mm, d273_d60_d51_d43 = 0 mm, d274_d61_d52 = 0 mm, d275_d62_d40 = 0 mm, d276_d63_d41 = 0 mm, d277_d64_d42 = 0 mm, d278_d65_d43 = 0 mm, d279_d40 = 0 mm, d280_d41 = 0 mm, d281_d42 = 0 mm, d282_d43 = 0 mm, d283_d118_d44 = 0 mm, d284_d119_d45 = 0 mm, d285_d120_d46_d44 = 0 mm, d286_d121_d47_d45 = 0 mm, d287_d122_d48_d40 = 0 mm, d288_d123_d49_d41 = 0 mm, d289_d124_d50_d42 = 0 mm, d290_d125_d51_d43 = 0 mm, d291_d126_d52 = 0 mm, d292_d127_d53_d44 = 0 mm, d293_d128_d54_d45 = 0 mm, d294_d129_d55_d46_d44 = 0 mm, d295_d130_d56_d47_d45 = 0 mm, d296_d131_d57_d48_d40 = 0 mm, d297_d132_d58_d49_d41 = 0 mm, d298_d133_d59_d50_d42 = 0 mm, d299_d134_d60_d51_d43 = 0 mm, d300_d135_d61_d52 = 0 mm, d301_d136_d62_d40 = 0 mm, d302_d137_d63_d41 = 0 mm, d303_d138_d64_d42 = 0 mm, d304_d139_d65_d43 = 0 mm, d305_d140_d40 = 0 mm, d306_d141_d41 = 0 mm, d307_d142_d42 = 0 mm, d308_d143_d43 = 0 mm, d309_d144_d66 = 0 mm, d310_d66 = 0 mm
